# Autodesk Inventor assembly: akf-60-nw25
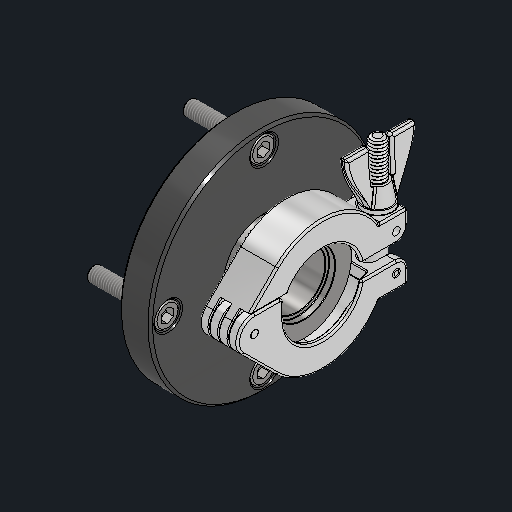
[picture p0: Inventor's stored thumbnail of the model, 512x512]
Saved by Autodesk Inventor 2026 (Build 300175050, 175E)
## iProperties
Created: 2025-12-20
Part Number: akf-60-nw25
Document SubType Name: Assembly
Designer: queezz
Author: queezz
## Documents named in this file (5)
- C:\Users\queezz\Dropbox\Drawings\PIHTI\PLD\akf-60-nw25.iam
- C:\Users\queezz\Dropbox\Drawings\PIHTI\PLD\nw-25-welded-30.ipt
- C:\Users\queezz\Dropbox\Drawings\PIHTI\ContentCenter\NW\NW25_clamp.ipt
- C:\Users\queezz\Dropbox\Drawings\PIHTI\PLD\akf-60-nw25.ipt
- C:\Users\queezz\Dropbox\Drawings\PIHTI\ContentCenter\Fastners\M6x25-SHCS.ipt
## Components (7 placed, 4 different names)
1. nw-25-welded-30:1
2. NW25_clamp:1
3. akf-60-nw25:1 — Rigid:2, Rigid:3, Rigid:4, Rigid:5
4. IS 2269 M6 x 25:1 — Rigid:4
5. IS 2269 M6 x 25:2 — Rigid:5
6. IS 2269 M6 x 25:3 — Rigid:3
7. IS 2269 M6 x 25:4 — Rigid:2
## Relationships (7: WeldJoint 5, Mate 2)
- [WeldJoint] (1 mm): nw-25-welded-30:1 ↔ akf-60-nw25:1
- [Mate]: nw-25-welded-30:1 ↔ NW25_clamp:1
- [Mate]: nw-25-welded-30:1 ↔ NW25_clamp:1
- Rigid:2 [WeldJoint]: akf-60-nw25:1 ↔ IS 2269 M6 x 25:4
- Rigid:3 [WeldJoint]: akf-60-nw25:1 ↔ IS 2269 M6 x 25:3
- Rigid:4 [WeldJoint]: akf-60-nw25:1 ↔ IS 2269 M6 x 25:1
- Rigid:5 [WeldJoint]: akf-60-nw25:1 ↔ IS 2269 M6 x 25:2
